# Autodesk Inventor assembly: A-2015
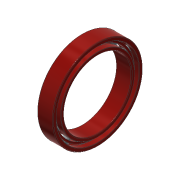
[picture p0: Inventor's stored thumbnail of the model, 180x180]
Saved by Autodesk Inventor 2019.4 (Build 234330000, 330)
## iProperties
Category: PARTsolutions
Company: NMB
Created: 2019-11-12
Part Number: A-2015
Catalog Web Link: www.cadenas.de
Description: Open type-
Vendor: NMB
Document SubType Name: Assembly
Designer: psadmin
Manufacturer: NMB
PSOL_IDENT_0: {$CADENAS_DATA\23d-libs\nmb\pbbp\radial_ball_bear_thin_secti\rbb_as\as_open_asmtab.prj},170 {VTYP=3D
PSOL_IDENT_1: },{STYP=ASSTAB},{NB=A-2015},{LINA=A-2015},{NN=Open type},{DATE=28.03.2019 02:31:01},{GEOMDATE=10.12.
PSOL_IDENT_2: 2013 03:09:46},{VERSION=},{LINEID=870},{WBVAR=},{WBNUMERIC=}  {NB=A-2015},{LINA=A-2015},{KT=DUMMY},{
PSOL_IDENT_3: IDNR=},{PN=A-2015},{SHLD=open},{FLANG=unflanged},{SD=15.000},{D=20.000},{B=3.500},{SR=0.15},{BCZ=14}
PSOL_IDENT_4: ,{DW=1.5875},{LI=16.40},{LO=18.43},{D1=0.000},{C1=0.00},{D2=0.0},{C2=0.00},{COR=582},{CR=944},{PCD=1
PSOL_IDENT_5: 7.500},{U=19.088},{W=15.913},{Y=0.794},{Z=0.794},{AA=0.000},{AC=0.00},{AD=0.000},{AF=0.00},{AQ=0.00}
PSOL_IDENT_6: ,{AH=0.00},{AI=0.00},{AJ=0.00},{PPATH=as_open_asmtpl.prj}
NN: Open type
NB: A-2015
NBSYN: $PN.
LINA: A-2015
PN: A-2015
SD: 15
D: 20
B: 3.5
SR: 0.15
BCZ: 14
DW: 1.5875
LI: 16.4
LO: 18.43
COR: 582
CR: 944
SUPPLIER: NMB
ARTICLENO: A-2015
BOMINFO: A-2015
CREATOR: CADENAS GmbH
Title: A-2015
Author: Cadenas PARTsolutions
## Documents named in this file (5)
- C:\Workspace\Yuni9\Inventor\Ref\DDA Series\NMB_A2015\A-2015.iam
- C:\Workspace\Yuni9\Inventor\Ref\DDA Series\NMB_A2015\A-2015_ir.ipt
- C:\Workspace\Yuni9\Inventor\Ref\DDA Series\NMB_A2015\A-2015_cage.ipt
- C:\Workspace\Yuni9\Inventor\Ref\DDA Series\NMB_A2015\A-2015_ball.ipt
- C:\Workspace\Yuni9\Inventor\Ref\DDA Series\NMB_A2015\A-2015_or.ipt
## Components (17 placed, 4 different names)
1. A-2015_ir:1
2. A-2015_cage:1
3. A-2015_or:1
4. A-2015_ball:1
5. A-2015_ball:2
6. A-2015_ball:3
7. A-2015_ball:4
8. A-2015_ball:5
9. A-2015_ball:6
10. A-2015_ball:7
11. A-2015_ball:8
12. A-2015_ball:9
13. A-2015_ball:10
14. A-2015_ball:11
15. A-2015_ball:12
16. A-2015_ball:13
17. A-2015_ball:14
## Component patterns: (14 elements, first: A-2015_ball:1)
